# Autodesk Inventor assembly: 回転軸フレーム
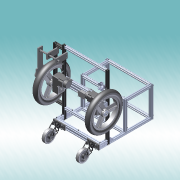
[picture p0: Inventor's stored thumbnail of the model, 180x180]
Saved by Autodesk Inventor 2015 (Build 190159000, 159)
## iProperties
Created: 2016-02-29
Part Number: 回転軸フレーム
Document SubType Name: Assembly
Designer: buzztaka
Author: buzztaka
## Documents named in this file (48)
- C:\Users\buzztaka\Downloads\2kk\回転軸フレーム.iam
- C:\Users\buzztaka\Downloads\2kk\wheel_12inch.ipt
- C:\Users\buzztaka\Downloads\2kk\motor shaft.ipt
- C:\Users\buzztaka\Downloads\2kk\machine key L1.ipt
- C:\Users\buzztaka\Downloads\2kk\machine key L2.ipt
- C:\Users\buzztaka\Downloads\2kk\motor part2.ipt
- C:\Users\buzztaka\Downloads\2kk\wheel-cap.ipt
- C:\Users\buzztaka\Downloads\2kk\kw\wheel-hub.ipt
- C:\Users\buzztaka\Downloads\2kk\caster.ipt
- C:\Users\buzztaka\Downloads\2kk\motor fix plate.ipt
- C:\Users\buzztaka\Downloads\2kk\spacer for caster.ipt
- C:\Users\buzztaka\Downloads\2kk\motor part1.ipt
- C:\Users\buzztaka\Downloads\2kk\Aluminum Extrusions2020-L2.ipt
- C:\Users\buzztaka\Downloads\2kk\Aluminum Extrusions2040-L2.ipt
- C:\Users\buzztaka\Downloads\2kk\Aluminum Extrusions2060-L2.ipt
- C:\Users\buzztaka\Downloads\2kk\Aluminum Extrusions2040-L3.ipt
- C:\Users\buzztaka\Downloads\2kk\Aluminum Extrusions2020-L4.ipt
- C:\Users\buzztaka\Downloads\2kk\Aluminum Extrusions2020-L5.ipt
- C:\Users\buzztaka\Downloads\2kk\Aluminum Extrusions2020-L6.ipt
- C:\Users\buzztaka\Downloads\2kk\Aluminum Extrusions2020-L7.ipt
- C:\Users\buzztaka\Downloads\2kk\hblfsn5.ipt
- C:\Users\buzztaka\Downloads\2kk\hblfsnf5.ipt
- C:\Users\buzztaka\Downloads\2kk\HBLFSSW5.ipt
- C:\Users\buzztaka\Downloads\2kk\hntaj5_5.ipt
- C:\Users\buzztaka\Downloads\2kk\Nat for Aluminum flame.ipt
- C:\Users\buzztaka\Downloads\2kk\Blind Joint Parts - Screw Joints.ipt
- C:\Users\buzztaka\Downloads\2kk\MTi-30.ipt
- C:\Users\buzztaka\Downloads\2kk\M5 washer.ipt
- C:\Users\buzztaka\Downloads\2kk\CapboltM5-10.ipt
- C:\Users\buzztaka\Downloads\2kk\CapboltM5-8.ipt
- C:\Users\buzztaka\Downloads\2kk\spring washer M5.ipt
- C:\Users\buzztaka\Downloads\2kk\spring washer M3.ipt
- C:\Users\buzztaka\Downloads\2kk\Capbolt-M3-6.ipt
- C:\Users\buzztaka\Downloads\2kk\CapboltM5-60.ipt
- C:\Users\buzztaka\Downloads\2kk\CapboltM6-10.ipt
- C:\Users\buzztaka\Downloads\2kk\M3ネジ16mm.ipt
- C:\Users\buzztaka\Downloads\2kk\washer M5.ipt
- C:\Users\buzztaka\Downloads\2kk\kw\HFSB5-2020-550-LCH-RWV-AH30-BH240-CH280-DH442-EH462.ipt
- C:\Users\buzztaka\Downloads\2kk\kw\HFSB5-2020-55-TPW.ipt
- C:\Users\buzztaka\Downloads\2kk\kw\HFSB5-2020-432-LCH-RCH-AH40-BH65.ipt
- C:\Users\buzztaka\Downloads\2kk\kw\HFSB5-2020-550-LCH-RWV-AH30-BH60-CH85-DH240-EH280-AP442.ipt
- C:\Users\buzztaka\Downloads\2kk\kw\C-SFL6901ZZ.ipt
- C:\Users\buzztaka\Downloads\2kk\回転軸取り付け板.ipt
- C:\Users\buzztaka\Downloads\2kk\回転軸.ipt
- C:\Users\buzztaka\Downloads\2kk\kw\タイヤアーム.ipt
- C:\Users\buzztaka\Downloads\2kk\kw\meh-30-pエンコーダ.ipt
- C:\Users\buzztaka\Downloads\2kk\kw\スプリングフランジ用ワッシャー（座金）.ipt
- C:\Users\buzztaka\Downloads\2kk\kw\スプリングフランジ0.1mm.ipt
## Components (258 placed, 47 different names)
1. wheel_12inch
2. motor shaft:1
3. machine key L1:1
4. machine key L2:1
5. motor part2:1
6. wheel-cap
7. wheel-hub
8. caster:1
9. motor fix plate:1
10. motor fix plate:2
11. spacer for caster:1
12. motor part1:1
13. spacer for caster:2
14. Aluminum Extrusions2020-L2:1
15. Aluminum Extrusions2040-L2:1
16. Aluminum Extrusions2060-L2:1 — 挿入:3, 挿入:4
17. Aluminum Extrusions2020-L2:2
18. Aluminum Extrusions2020-L2:3
19. Aluminum Extrusions2020-L2:4
20. Aluminum Extrusions2020-L2:5
21. Aluminum Extrusions2020-L2:6
22. Aluminum Extrusions2040-L3:1
23. Aluminum Extrusions2020-L4:1
24. Aluminum Extrusions2020-L5:1
25. Aluminum Extrusions2020-L6:1
26. Aluminum Extrusions2020-L7:1
27. hblfsn5
28. hblfsnf5:1
29. hblfsnf5:2
30. HBLFSSW5
31. hntaj5_5:1
32. hntaj5_5:2
33. Nat for Aluminum flame:1
34. Nat for Aluminum flame:2
35. Nat for Aluminum flame:3
36. Nat for Aluminum flame:4
37. hntaj5_5:3
38. hntaj5_5:4
39. hntaj5_5:5
40. hntaj5_5:6
41. hntaj5_5:12
42. Nat for Aluminum flame:5
43. Blind Joint Parts - Screw Joints:1
44. Blind Joint Parts - Screw Joints:2
45. Blind Joint Parts - Screw Joints:3
46. Blind Joint Parts - Screw Joints:4
47. Blind Joint Parts - Screw Joints:5
48. Blind Joint Parts - Screw Joints:6
49. Blind Joint Parts - Screw Joints:7
50. Blind Joint Parts - Screw Joints:8
51. Blind Joint Parts - Screw Joints:9
52. Blind Joint Parts - Screw Joints:10
53. Nat for Aluminum flame:6
54. Nat for Aluminum flame:7
55. Nat for Aluminum flame:8
56. Nat for Aluminum flame:9
57. Nat for Aluminum flame:10
58. Nat for Aluminum flame:11
59. Nat for Aluminum flame:12
60. Nat for Aluminum flame:13
61. Nat for Aluminum flame:14
62. hntaj5_5:16
63. hntaj5_5:17
64. hntaj5_5:18
65. hntaj5_5:19
66. hntaj5_5:20
67. hntaj5_5:21
68. hntaj5_5:22
69. hntaj5_5:23
70. Blind Joint Parts - Screw Joints:11
71. Blind Joint Parts - Screw Joints:12
72. hntaj5_5:24
73. hntaj5_5:25
74. caster:2
75. Aluminum Extrusions2040-L3:2
76. wheel_12inch:1
77. motor fix plate:3
78. motor fix plate:4
79. wheel-cap:1
80. machine key L2:2
81. motor shaft:2
82. machine key L1:2
83. wheel-hub:1
84. MTi-30
85. Aluminum Extrusions2020-L4:2
86. Aluminum Extrusions2020-L5:2
87. hblfsn5:1
88. Aluminum Extrusions2020-L6:2
89. Aluminum Extrusions2020-L7:2
90. CapboltM5-10:2
91. CapboltM5-10:3
92. CapboltM5-10:4
93. CapboltM5-10:5
94. CapboltM5-8:1
95. CapboltM5-8:2
96. CapboltM5-10:6
97. CapboltM5-10:7
98. CapboltM5-10:8
99. CapboltM5-10:9
100. CapboltM5-10:12
101. CapboltM5-10:13
102. CapboltM5-8:6
103. CapboltM5-8:7
104. CapboltM5-8:8
105. CapboltM5-10:14
106. CapboltM5-10:15
107. CapboltM5-10:16
108. CapboltM5-10:17
109. CapboltM5-10:18
110. CapboltM5-10:19
111. CapboltM5-8:12
112. spring washer M5:4
113. CapboltM5-8:13
114. spring washer M5:5
115. Capbolt-M3-6:3
116. spring washer M3:3
117. CapboltM5-60:1
118. CapboltM6-10:1
119. M3ネジ16mm:1
120. washer M5:1
121. spring washer M5:6
122. M5 washer:2
123. washer M5:2
124. CapboltM5-8:14
125. spring washer M5:7
126. CapboltM5-8:15
127. spring washer M5:8
128. M5 washer:3
129. CapboltM5-60:2
130. spring washer M5:9
131. CapboltM5-10:20
132. CapboltM5-8:16
133. spring washer M5:10
134. CapboltM5-8:17
135. spring washer M5:11
136. CapboltM5-8:18
137. spring washer M5:12
138. CapboltM5-8:19
139. spring washer M5:13
140. CapboltM5-8:20
141. spring washer M5:14
142. CapboltM5-8:21
143. spring washer M5:15
144. hblfsnf5:3
145. Blind Joint Parts - Screw Joints:16
146. Blind Joint Parts - Screw Joints:17
147. Blind Joint Parts - Screw Joints:18
148. Blind Joint Parts - Screw Joints:19
149. hntaj5_5:26
150. CapboltM5-10:21
151. CapboltM5-10:22
152. Nat for Aluminum flame:15
153. Blind Joint Parts - Screw Joints:20
154. Blind Joint Parts - Screw Joints:21
155. Nat for Aluminum flame:16
156. CapboltM5-8:22
157. Nat for Aluminum flame:17
158. CapboltM5-8:23
159. hntaj5_5:27
160. CapboltM5-10:23
161. hntaj5_5:28
162. CapboltM5-10:24
163. Blind Joint Parts - Screw Joints:22
164. Blind Joint Parts - Screw Joints:23
165. Blind Joint Parts - Screw Joints:24
166. Blind Joint Parts - Screw Joints:25
167. Nat for Aluminum flame:18
168. CapboltM5-10:27
169. CapboltM5-10:28
170. Nat for Aluminum flame:19
171. Nat for Aluminum flame:20
172. CapboltM5-10:29
173. Nat for Aluminum flame:21
174. CapboltM5-10:30
175. Nat for Aluminum flame:22
176. CapboltM5-10:31
177. CapboltM5-10:32
178. Nat for Aluminum flame:23
179. spring washer M3:13
180. spring washer M3:14
181. Capbolt-M3-6:13
182. Capbolt-M3-6:14
183. CapboltM6-10:2
184. CapboltM6-10:3
185. CapboltM6-10:4
186. CapboltM5-10:33
187. CapboltM5-10:34
188. CapboltM5-10:35
189. CapboltM5-10:36
190. CapboltM5-10:37
191. CapboltM6-10:5
192. CapboltM6-10:6
193. CapboltM6-10:7
194. CapboltM6-10:8
195. CapboltM5-10:38
196. CapboltM5-10:39
197. M3ネジ16mm:2
198. M3ネジ16mm:3
199. M3ネジ16mm:4
200. hntaj5_5:35
201. Blind Joint Parts - Screw Joints:26
202. CapboltM5-8:28
203. spring washer M5:17
204. CapboltM5-8:29
205. spring washer M5:18
206. hntaj5_5:36
207. CapboltM5-8:30
208. spring washer M5:19
209. hntaj5_5:37
210. hntaj5_5:38
211. CapboltM5-8:31
212. spring washer M5:20
213. washer M5:3
214. CapboltM5-8:32
215. spring washer M5:21
216. M3ネジ16mm:5
217. M3ネジ16mm:6
218. M3ネジ16mm:7
219. CapboltM5-60:3
220. spring washer M5:22
221. M3ネジ16mm:8
222. spring washer M5:23
223. CapboltM5-60:4
224. CapboltM5-8:33
225. washer M5:4
226. M5 washer:4
227. M5 washer:5
228. hntaj5_5:39
229. CapboltM5-8:34
230. spring washer M5:24
231. CapboltM5-8:35
232. spring washer M5:25
233. hntaj5_5:40
234. CapboltM5-8:36
235. spring washer M5:26
236. hntaj5_5:42
237. hntaj5_5:42
238. spring washer M5:27
239. CapboltM5-8:37
240. spring washer M5:28
241. HFSB5-2020-550-LCH-RWV-AH30-BH240-CH280-DH442-EH462:2 — 挿入:3, 挿入:4
242. HFSB5-2020-55-TPW:1 — 挿入:26, 挿入:29
243. HFSB5-2020-55-TPW:2 — 挿入:27, 挿入:28
244. HFSB5-2020-550-LCH-RWV-AH30-BH60-CH85-DH240-EH280-AP442:1 — 挿入:26, 挿入:27, 挿入:32, 挿入:33
245. HFSB5-2020-432-LCH-RCH-AH40-BH65:1 — 挿入:28, 挿入:29, 挿入:37, 挿入:38
246. C-SFL6901ZZ:2 — 挿入:39
247. 回転軸取り付け板:2 — 挿入:32, 挿入:33
248. C-SFL6901ZZ:3
249. 回転軸取り付け板:3 — 挿入:37, 挿入:38
250. 回転軸:1 — 挿入:39, 挿入:41
251. C-SFL6901ZZ:4 — 挿入:40, 挿入:41
252. タイヤアーム:1 — 挿入:40, 挿入:42, 挿入:48, 挿入:49
253. C-SFL6901ZZ:5 — 挿入:42
254. meh-30-pエンコーダ:1
255. スプリングフランジ用ワッシャー（座金）:1
256. スプリングフランジ用ワッシャー（座金）:2
257. スプリングフランジ用ワッシャー（座金）:3
258. スプリングフランジ0.1mm:1 — 挿入:48, 挿入:49
## Relationships (25: Insert 25)
- 挿入:3 [Insert]: Aluminum Extrusions2060-L2:1 ↔ HFSB5-2020-550-LCH-RWV-AH30-BH240-CH280-DH442-EH462:2
- 挿入:4 [Insert]: Aluminum Extrusions2060-L2:1 ↔ HFSB5-2020-550-LCH-RWV-AH30-BH240-CH280-DH442-EH462:2
- [Insert]: Aluminum Extrusions2020-L2:1 ↔ HFSB5-2020-550-LCH-RWV-AH30-BH60-CH85-DH240-EH280-AP442:1
- [Insert]: Aluminum Extrusions2060-L2:1 ↔ HFSB5-2020-550-LCH-RWV-AH30-BH60-CH85-DH240-EH280-AP442:1
- 挿入:26 [Insert]: HFSB5-2020-55-TPW:1 ↔ HFSB5-2020-550-LCH-RWV-AH30-BH60-CH85-DH240-EH280-AP442:1
- 挿入:27 [Insert]: HFSB5-2020-55-TPW:2 ↔ HFSB5-2020-550-LCH-RWV-AH30-BH60-CH85-DH240-EH280-AP442:1
- 挿入:28 [Insert]: HFSB5-2020-55-TPW:2 ↔ HFSB5-2020-432-LCH-RCH-AH40-BH65:1
- 挿入:29 [Insert]: HFSB5-2020-55-TPW:1 ↔ HFSB5-2020-432-LCH-RCH-AH40-BH65:1
- [Insert]: C-SFL6901ZZ:2 ↔ 回転軸取り付け板:2
- 挿入:32 [Insert]: HFSB5-2020-550-LCH-RWV-AH30-BH60-CH85-DH240-EH280-AP442:1 ↔ 回転軸取り付け板:2
- 挿入:33 [Insert]: HFSB5-2020-550-LCH-RWV-AH30-BH60-CH85-DH240-EH280-AP442:1 ↔ 回転軸取り付け板:2
- [Insert]: C-SFL6901ZZ:3 ↔ 回転軸取り付け板:3
- 挿入:37 [Insert]: HFSB5-2020-432-LCH-RCH-AH40-BH65:1 ↔ 回転軸取り付け板:3
- 挿入:38 [Insert]: HFSB5-2020-432-LCH-RCH-AH40-BH65:1 ↔ 回転軸取り付け板:3
- 挿入:39 [Insert] (-20 mm): C-SFL6901ZZ:2 ↔ 回転軸:1
- 挿入:40 [Insert]: C-SFL6901ZZ:4 ↔ タイヤアーム:1
- 挿入:41 [Insert] (-10 mm): 回転軸:1 ↔ C-SFL6901ZZ:4
- 挿入:42 [Insert]: タイヤアーム:1 ↔ C-SFL6901ZZ:5
- [Insert]: meh-30-pエンコーダ:1 ↔ スプリングフランジ用ワッシャー（座金）:2
- [Insert]: meh-30-pエンコーダ:1 ↔ スプリングフランジ用ワッシャー（座金）:1
- [Insert]: meh-30-pエンコーダ:1 ↔ スプリングフランジ用ワッシャー（座金）:3
- [Insert]: スプリングフランジ用ワッシャー（座金）:2 ↔ スプリングフランジ0.1mm:1
- [Insert]: スプリングフランジ用ワッシャー（座金）:3 ↔ スプリングフランジ0.1mm:1
- 挿入:48 [Insert]: タイヤアーム:1 ↔ スプリングフランジ0.1mm:1
- 挿入:49 [Insert]: タイヤアーム:1 ↔ スプリングフランジ0.1mm:1
## Named parameters: d53_d52 = 0 mm, d58_d52 = 0 mm
